# Autodesk Inventor assembly: leg_assembly
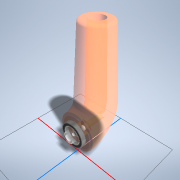
[picture p0: Inventor's stored thumbnail of the model, 180x180]
Saved by Autodesk Inventor 2020.2 (Build 242310000, 310)
## iProperties
Created: 2020-10-23
Part Number: leg_assembly
Document SubType Name: Assembly
Designer: boxi
Author: boxi
## Documents named in this file (6)
- C:\Users\boxi\Documents\flexipod_hardware\mechanical_model\leg_assembly.iam
- C:\Users\boxi\Documents\flexipod_hardware\mechanical_model\leg.ipt
- C:\Users\boxi\Documents\flexipod_hardware\mechanical_model\leg_coupler.ipt
- leg_coupler.ipt
- C:\Users\boxi\Documents\flexipod_hardware\mechanical_model\bearing_6806_2RS_30x42x7.ipt
- C:\Users\boxi\Documents\flexipod_hardware\mechanical_model\Screw GB_T 70.1 M5 x 16.ipt
## Components (4 placed, 4 different names)
1. leg:1 — Rigid:1
2. leg_coupler:1 — Rigid:1, Rigid:2, Rigid:3
3. bearing_6806_2RS_30x42x7:1 — Rigid:2
4. Screw GB_T 70.1 M5 x 16:1 — Rigid:3
## Relationships (3: WeldJoint 3)
- Rigid:1 [WeldJoint]: leg:1 ↔ leg_coupler:1
- Rigid:2 [WeldJoint]: leg_coupler:1 ↔ bearing_6806_2RS_30x42x7:1
- Rigid:3 [WeldJoint]: leg_coupler:1 ↔ Screw GB_T 70.1 M5 x 16:1
